# Autodesk Inventor assembly: Assy
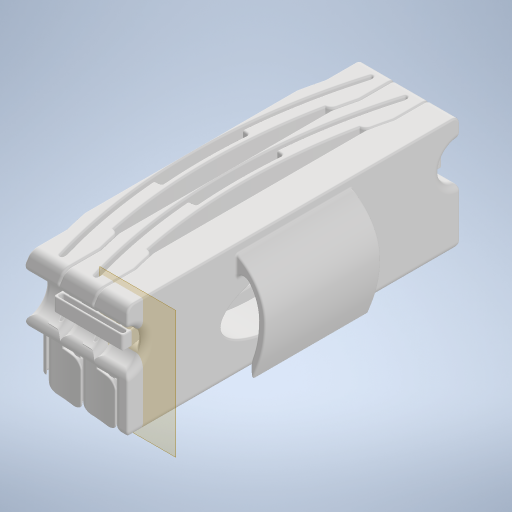
[picture p0: Inventor's stored thumbnail of the model, 512x512]
Saved by Autodesk Inventor 2024 (Build 280153000, 153)
## iProperties
Created: 2024-12-25
Part Number: Assy
Document SubType Name: Assembly
Designer: rrenkit
Author: rrenkit
## Documents named in this file (4)
- C:\Users\rrenkit\Documents\CAD\Clip-On Sunglasses Holder\V2\Assy.iam
- C:\Users\rrenkit\Documents\CAD\Clip-On Sunglasses Holder\V2\housing.ipt
- C:\Users\rrenkit\Documents\CAD\Clip-On Sunglasses Holder\V2\clip.ipt
- C:\Users\rrenkit\Documents\CAD\Clip-On Sunglasses Holder\V2\bracket.ipt
## Components (5 placed, 3 different names)
1. housing:1 — Mate:1, Flush:1, Mate:2
2. housing:2 — Mate:1, Flush:1, Mate:2, Mate:3, Mate:4, Mate:5
3. clip:1 — Mate:3, Mate:4, Mate:5, Mate:6, Mate:7, Mate:8, Mate:9, Mate:10, Mate:11
4. bracket:1 — Mate:6, Mate:7, Mate:8
5. bracket:2 — Mate:9, Mate:10, Mate:11
## Relationships (12: Mate 11, Flush 1)
- Mate:1: housing:1 ↔ housing:2
- Flush:1: housing:1 ↔ housing:2
- Mate:2: housing:1 ↔ housing:2
- Mate:3: housing:2 ↔ clip:1
- Mate:4: housing:2 ↔ clip:1
- Mate:5: housing:2 ↔ clip:1
- Mate:6: clip:1 ↔ bracket:1
- Mate:7: clip:1 ↔ bracket:1
- Mate:8: clip:1 ↔ bracket:1
- Mate:9: clip:1 ↔ bracket:2
- Mate:10: clip:1 ↔ bracket:2
- Mate:11: clip:1 ↔ bracket:2
